# Autodesk Inventor assembly: single head
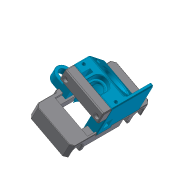
[picture p0: Inventor's stored thumbnail of the model, 180x180]
Saved by Autodesk Inventor 2015 (Build 190159000, 159)
## iProperties
Created: 2020-04-10
Part Number: single head
Document SubType Name: Assembly
Designer: Ghassan Yusuf
Author: Ghassan Yusuf
## Documents named in this file (5)
- X:\TAKEONE\Products\takeone-3D-printer\model\3D\single head.iam
- X:\TAKEONE\Products\takeone-3D-printer\model\3D\Extruder Heat Sink.ipt
- X:\TAKEONE\Products\takeone-3D-printer\model\3D\Hotend Holder & Vent.ipt
- X:\TAKEONE\Products\takeone-3D-printer\model\3D\Single Extruder Carriage.ipt
- X:\TAKEONE\Products\takeone-3D-printer\model\3D\single extruder securer.ipt
## Components (4 placed, 4 different names)
1. Extruder Heat Sink:1 — Insert:1
2. Hotend Holder & Vent:1 — Insert:1, Mate:1, Flush:1, Mate:2, Insert:2, Insert:3
3. Single Extruder Carriage:1 — Mate:1, Flush:1, Mate:2
4. single extruder securer:1 — Insert:2, Insert:3
## Relationships (6: Insert 3, Mate 2, Flush 1)
- Insert:1: Extruder Heat Sink:1 ↔ Hotend Holder & Vent:1
- Mate:1: Hotend Holder & Vent:1 ↔ Single Extruder Carriage:1
- Flush:1: Hotend Holder & Vent:1 ↔ Single Extruder Carriage:1
- Mate:2 (0.1 mm): Hotend Holder & Vent:1 ↔ Single Extruder Carriage:1
- Insert:2: Hotend Holder & Vent:1 ↔ single extruder securer:1
- Insert:3: Hotend Holder & Vent:1 ↔ single extruder securer:1
